# Autodesk Inventor assembly: rotary control
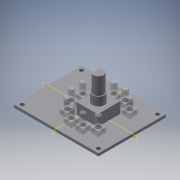
[picture p0: Inventor's stored thumbnail of the model, 180x180]
Saved by Autodesk Inventor 2016 (Build 200138000, 138)
## iProperties
Created: 2015-10-20
Part Number: rotary control
Document SubType Name: Assembly
Designer: jeremyhale
Author: jeremyhale
## Documents named in this file (4)
- \\psf\Home\Documents\Poorhouse\git\p0001\rotary control.iam
- \\psf\Home\Documents\Poorhouse\git\p0001\pcb rotary control.ipt
- \\psf\Home\Documents\Poorhouse\git\p0001\VLP-350-F.ipt
- \\psf\Home\Documents\Poorhouse\git\p0001\PEC11R-4215F-S0024.ipt
## Components (12 placed, 3 different names)
1. pcb rotary control:1 — Rotational:1, Rotational:2, Rotational:3, Rotational:4, Rotational:5, Rotational:6, Rotational:7, Rotational:8, Rotational:9, Rotational:10, Rotational:11, Rotational:12, Rotational:13, Rotational:14, Rotational:15, Rotational:16, Rotational:17, Rotational:18, Rotational:19, Rotational:20, Rigid:1
2. VLP-350-F:1 — Rotational:1, Rotational:2
3. VLP-350-F:2 — Rotational:3, Rotational:4
4. VLP-350-F:3 — Rotational:5, Rotational:6
5. VLP-350-F:4 — Rotational:7, Rotational:8
6. VLP-350-F:5 — Rotational:13, Rotational:14
7. VLP-350-F:6 — Rotational:15, Rotational:16
8. VLP-350-F:7 — Rotational:17, Rotational:18
9. VLP-350-F:8 — Rotational:19, Rotational:20
10. VLP-350-F:9 — Rotational:11, Rotational:12
11. VLP-350-F:10 — Rotational:9, Rotational:10
12. PEC11R-4215F-S0024:1 — Rigid:1
## Relationships (21: RevoluteJoint 20, WeldJoint 1)
- Rotational:1 [RevoluteJoint]: pcb rotary control:1 ↔ VLP-350-F:1
- Rotational:2 [RevoluteJoint]: pcb rotary control:1 ↔ VLP-350-F:1
- Rotational:3 [RevoluteJoint]: pcb rotary control:1 ↔ VLP-350-F:2
- Rotational:4 [RevoluteJoint]: pcb rotary control:1 ↔ VLP-350-F:2
- Rotational:5 [RevoluteJoint]: pcb rotary control:1 ↔ VLP-350-F:3
- Rotational:6 [RevoluteJoint]: pcb rotary control:1 ↔ VLP-350-F:3
- Rotational:7 [RevoluteJoint]: pcb rotary control:1 ↔ VLP-350-F:4
- Rotational:8 [RevoluteJoint]: pcb rotary control:1 ↔ VLP-350-F:4
- Rotational:9 [RevoluteJoint]: pcb rotary control:1 ↔ VLP-350-F:10
- Rotational:10 [RevoluteJoint]: pcb rotary control:1 ↔ VLP-350-F:10
- Rotational:11 [RevoluteJoint]: pcb rotary control:1 ↔ VLP-350-F:9
- Rotational:12 [RevoluteJoint]: pcb rotary control:1 ↔ VLP-350-F:9
- Rotational:13 [RevoluteJoint]: pcb rotary control:1 ↔ VLP-350-F:5
- Rotational:14 [RevoluteJoint]: pcb rotary control:1 ↔ VLP-350-F:5
- Rotational:15 [RevoluteJoint]: pcb rotary control:1 ↔ VLP-350-F:6
- Rotational:16 [RevoluteJoint]: pcb rotary control:1 ↔ VLP-350-F:6
- Rotational:17 [RevoluteJoint]: pcb rotary control:1 ↔ VLP-350-F:7
- Rotational:18 [RevoluteJoint]: pcb rotary control:1 ↔ VLP-350-F:7
- Rotational:19 [RevoluteJoint]: pcb rotary control:1 ↔ VLP-350-F:8
- Rotational:20 [RevoluteJoint]: pcb rotary control:1 ↔ VLP-350-F:8
- Rigid:1 [WeldJoint]: pcb rotary control:1 ↔ PEC11R-4215F-S0024:1
